# Autodesk Inventor assembly: Assembly2
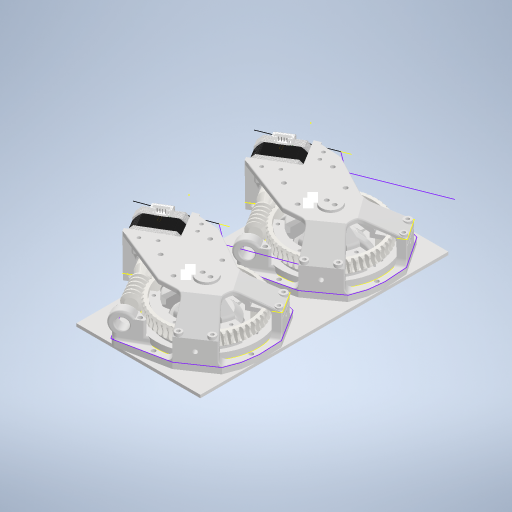
[picture p0: Inventor's stored thumbnail of the model, 512x512]
Saved by Autodesk Inventor 2023.1 (Build 271208000, 208)
## iProperties
Created: 2022-12-26
Part Number: Assembly2
Document SubType Name: Assembly
Designer: USER
Author: USER
## Documents named in this file (4)
- D:\Assembly2.iam
- D:\knob_holder.ipt
- D:\Plate.ipt
- D:\Assembly1.iam
## Components (5 placed, 3 different names)
1. knob_holder:1 — Mate:2, Mate:4, Mate:6
2. Plate:1 — Mate:1, Mate:2, Mate:3, Mate:4, Mate:5, Mate:7
3. knob_holder:2 — Mate:1, Mate:3, Mate:8
4. Assembly1:1 [sub-assembly] — Mate:5, Mate:6
5. Assembly1:2 [sub-assembly] — Mate:7, Mate:8
## Relationships (8: Mate 8)
- Mate:1: Plate:1 ↔ knob_holder:2
- Mate:2: knob_holder:1 ↔ Plate:1
- Mate:3: Plate:1 ↔ knob_holder:2
- Mate:4: knob_holder:1 ↔ Plate:1
- Mate:5: Plate:1 ↔ Assembly1:1
- Mate:6: knob_holder:1 ↔ Assembly1:1
- Mate:7: Plate:1 ↔ Assembly1:2
- Mate:8: knob_holder:2 ↔ Assembly1:2
